# Autodesk Inventor assembly: face_cborka_2
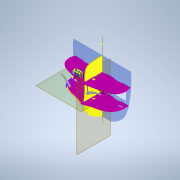
[picture p0: Inventor's stored thumbnail of the model, 180x180]
Saved by Autodesk Inventor 2020 (Build 240168000, 168)
## iProperties
Created: 2022-02-15
Part Number: face_cborka_2
Document SubType Name: Assembly
Designer: Администратор
Author: Администратор
## Documents named in this file (9)
- \\sch239.net\UserHomes\Students\25\2\polubutkinaaa.25\OnStage\face_cborka\Лицо_пересборка\face_cborka_2.iam
- \\sch239.net\UserHomes\Students\25\2\polubutkinaaa.25\OnStage\face_cborka\Лицо_пересборка\mesh_face_front_1.ipt
- \\sch239.net\UserHomes\Students\25\2\polubutkinaaa.25\OnStage\face_cborka\Лицо_пересборка\Глаз\Face 2.0 full\платформа_глаза.ipt
- \\sch239.net\UserHomes\Students\25\2\polubutkinaaa.25\OnStage\face_cborka\Лицо_пересборка\Глаз\Face 2.0 full\head_1.ipt
- \\sch239.net\UserHomes\Students\25\2\polubutkinaaa.25\OnStage\face_cborka\Лицо_пересборка\бровь.ipt
- \\sch239.net\UserHomes\Students\25\2\polubutkinaaa.25\OnStage\face_cborka\Лицо_пересборка\платформа_для_бровей.ipt
- \\sch239.net\UserHomes\Students\25\2\polubutkinaaa.25\OnStage\face_cborka\Лицо_пересборка\поперечная_поддержка.ipt
- \\sch239.net\UserHomes\Students\25\2\polubutkinaaa.25\OnStage\face_cborka\Лицо_пересборка\сборка_держатель_серво_брови.iam
- \\sch239.net\UserHomes\Students\25\2\polubutkinaaa.25\OnStage\face_cborka\Лицо_пересборка\ard_uno_r3.ipt
## Components (9 placed, 8 different names)
1. head_1:1 — Совмещение:2, Совмещение:4, Совмещение:10, Заподлицо:10, Совмещение:34
2. mesh_face_front_1:1 — Совмещение:4, Заподлицо:2, Заподлицо:3, Заподлицо:4, Совмещение:6, Заподлицо:5
3. платформа_глаза:1 — Совмещение:6, Заподлицо:5, Заподлицо:10, Симметрия:1, Совмещение:14, Угол:3, Совмещение:17, Совмещение:18, Совмещение:22, Совмещение:23
4. бровь:1 — Совмещение:33
5. бровь:2
6. платформа_для_бровей:1 — Совмещение:19, Совмещение:20, Совмещение:26, Совмещение:27, Совмещение:30
7. поперечная_поддержка:1 — Заподлицо:12, Заподлицо:13, Симметрия:1, Совмещение:13, Угол:2, Совмещение:15
8. сборка_держатель_серво_брови:1 [sub-assembly] — Совмещение:28, Совмещение:29
9. ard_uno_r3:1 — Совмещение:34
## Relationships (33: Mate 22, Flush 7, Angle 3, Symmetry 1)
- Совмещение:2 [Mate]: head_1:1
- Совмещение:4 [Mate]: head_1:1 ↔ mesh_face_front_1:1
- Заподлицо:2 [Flush] (40 mm): mesh_face_front_1:1
- Заподлицо:3 [Flush]: mesh_face_front_1:1
- Заподлицо:4 [Flush]: mesh_face_front_1:1
- Совмещение:6 [Mate]: mesh_face_front_1:1 ↔ платформа_глаза:1
- Заподлицо:5 [Flush] (-14 mm): mesh_face_front_1:1 ↔ платформа_глаза:1
- Совмещение:10 [Mate] (206 mm): head_1:1
- Заподлицо:10 [Flush]: head_1:1 ↔ платформа_глаза:1
- Заподлицо:12 [Flush]: поперечная_поддержка:1
- Заподлицо:13 [Flush]: поперечная_поддержка:1
- Симметрия:1 [Symmetry]: платформа_глаза:1 ↔ поперечная_поддержка:1
- Совмещение:13 [Mate]: поперечная_поддержка:1
- Угол:2 [Angle] (90 deg): поперечная_поддержка:1
- Совмещение:14 [Mate]: платформа_глаза:1
- Угол:3 [Angle] (180 deg): платформа_глаза:1
- Совмещение:15 [Mate]: поперечная_поддержка:1
- Угол:4 [Angle] (180 deg)
- Совмещение:16 [Mate]
- Совмещение:17 [Mate]: платформа_глаза:1
- Совмещение:18 [Mate]: платформа_глаза:1
- Совмещение:19 [Mate]: платформа_для_бровей:1
- Совмещение:20 [Mate]: платформа_для_бровей:1
- Совмещение:21 [Mate]
- Совмещение:22 [Mate]: платформа_глаза:1
- Совмещение:23 [Mate]: платформа_глаза:1
- Совмещение:26 [Mate]: платформа_для_бровей:1
- Совмещение:27 [Mate]: платформа_для_бровей:1
- Совмещение:28 [Mate]: сборка_держатель_серво_брови:1
- Совмещение:29 [Mate]: сборка_держатель_серво_брови:1
- Совмещение:30 [Mate]: платформа_для_бровей:1
- Совмещение:33 [Mate]: бровь:1
- Совмещение:34 [Mate]: head_1:1 ↔ ard_uno_r3:1
